# Autodesk Inventor assembly: 4x2020_encoder
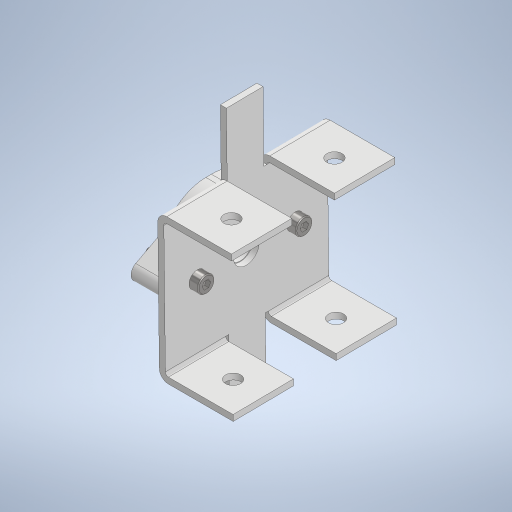
[picture p0: Inventor's stored thumbnail of the model, 512x512]
Saved by Autodesk Inventor 2024 (Build 280153000, 153)
## iProperties
Created: 2025-12-17
Part Number: 4x2020_encoder
Document SubType Name: Assembly
Designer: schar
Author: schar
## Documents named in this file (5)
- C:\Users\schar\Desktop\projectBlueprint\AMSTS\hardware\4x2020_encoder.iam
- C:\Users\schar\Desktop\projectBlueprint\AMSTS\hardware\4x2020_blank.ipt
- C:\Users\schar\Desktop\projectBlueprint\AMSTS\hardware\AMT102-0512-I5000-5.ipt
- C:\Users\schar\Documents\Inventor\Content Center Files\R2024\en-US\AS 1420\AS 1420 - 1973 - M3 x 16.ipt
- C:\Users\schar\Documents\Inventor\Content Center Files\R2024\en-US\ISO 4032(1)\ISO 4032 - M2,5DIN EN.ipt
## Components (6 placed, 4 different names)
1. 4x2020_blank:1 — Mate:4, Mate:5, Mate:7, Mate:8, Mate:9
2. AMT102-0512-I5000-5:1 — Insert:1, Insert:2, Mate:6, Mate:7
3. AS 1420 - Metric M3 x 16:1 — Mate:6, Mate:8, Mate:9
4. AS 1420 - Metric M3 x 16:2 — Mate:4, Mate:5
5. DIN EN 24032 M2,5:1 — Insert:1
6. DIN EN 24032 M2,5:2 — Insert:2
## Relationships (8: Mate 6, Insert 2)
- Mate:4: 4x2020_blank:1 ↔ AS 1420 - Metric M3 x 16:2
- Mate:5: 4x2020_blank:1 ↔ AS 1420 - Metric M3 x 16:2
- Insert:1: AMT102-0512-I5000-5:1 ↔ DIN EN 24032 M2,5:1
- Insert:2: AMT102-0512-I5000-5:1 ↔ DIN EN 24032 M2,5:2
- Mate:6: AMT102-0512-I5000-5:1 ↔ AS 1420 - Metric M3 x 16:1
- Mate:7: 4x2020_blank:1 ↔ AMT102-0512-I5000-5:1
- Mate:8: 4x2020_blank:1 ↔ AS 1420 - Metric M3 x 16:1
- Mate:9: 4x2020_blank:1 ↔ AS 1420 - Metric M3 x 16:1
